# Autodesk Inventor assembly: ensamble
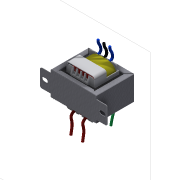
[picture p0: Inventor's stored thumbnail of the model, 180x180]
Saved by Autodesk Inventor 2016 (Build 200138000, 138)
## iProperties
Created: 2017-03-04
Part Number: ensamble
Document SubType Name: Assembly
Designer: julianesteban
Author: julianesteban
## Documents named in this file (3)
- C:\Users\julianesteban\Google Drive\Julian y Espitia\diseños inventor elementos comerciales\transformador\ensamble.iam
- C:\Users\julianesteban\Google Drive\Julian y Espitia\diseños inventor elementos comerciales\transformador\transformador 2.ipt
- C:\Users\julianesteban\Google Drive\Julian y Espitia\diseños inventor elementos comerciales\transformador\transformador.ipt
## Components (2 placed, 2 different names)
1. transformador 2:1 — Mate:1, Flush:1, Flush:2
2. transformador:1 — Mate:1, Flush:1, Flush:2
## Relationships (3: Flush 2, Mate 1)
- Mate:1: transformador 2:1 ↔ transformador:1
- Flush:1: transformador 2:1 ↔ transformador:1
- Flush:2: transformador 2:1 ↔ transformador:1
